# Autodesk Inventor assembly: 100027
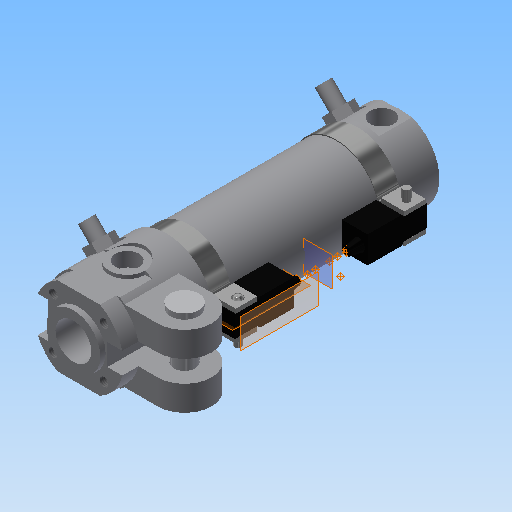
[picture p0: Inventor's stored thumbnail of the model, 512x512]
Saved by Autodesk Inventor 2020.1 (Build 241239000, 239)
## iProperties
Company: AUTODESK, INC.
Part Number: 100027
Document SubType Name: Assembly
Created: 2003-06-25
Designer: SCHNEIDER K.
Description: 70mm STROKE
Project: ADSK-000-000000
Control State: 0
Master: False
Checked Out: False
Shininess: 64.0
Length Units: 11269
Angle Units: 11279
Time Units: 11290
Mass Units: 11283
Length Display Precision: 2
Angle Display Precision: 2
Compacted: True
Stroke: 70.00 mm
Density: 0.0
Volumn: 0.0
Area: 0.0
PropertySet Name: Model Information
Title: PH CYLINDER
Author: schneik
Revision Number: -
## Documents named in this file (5)
- C:\Users\thom_tremblay\Desktop\Inventor ACP Data\Assemblies\PH-000-001.iam
- C:\Users\thom_tremblay\Desktop\Inventor ACP Data\Parts\PH-200-012.ipt
- C:\Users\thom_tremblay\Desktop\Inventor ACP Data\Parts\PH-200-010.ipt
- C:\Users\thom_tremblay\Desktop\Inventor ACP Data\Parts\PH-200-011.ipt
- C:\Users\thom_tremblay\Desktop\Inventor ACP Data\Parts\PH-200-014.ipt
## Components (6 placed, 4 different names)
1. PH-200-012:1 — Insert:6, Insert:7, Insert:4, Angle:4, Angle:5
2. PH-200-010:1 — Insert:1, Angle:1, Flush:1, Flush:2, Flush:3
3. PH-200-010:2 — Insert:2, Angle:2
4. PH-200-011:1 — Insert:6, Insert:1, Angle:1, Angle:4
5. PH-200-011:2 — Insert:7, Insert:2, Angle:2, Angle:5
6. PH-200-014:1 — Insert:4
## Relationships (15: Insert 5, Angle 4, Flush 3, Mate 3)
- Insert:6 (0.5 mm): PH-200-012:1 ↔ PH-200-011:1
- Insert:7 (23.5 mm): PH-200-012:1 ↔ PH-200-011:2
- Insert:1: PH-200-010:1 ↔ PH-200-011:1
- Angle:1 (0 deg): PH-200-010:1 ↔ PH-200-011:1
- Insert:2: PH-200-010:2 ↔ PH-200-011:2
- Angle:2 (0 deg): PH-200-010:2 ↔ PH-200-011:2
- Insert:4: PH-200-012:1 ↔ PH-200-014:1
- Angle:4 (180 deg): PH-200-012:1 ↔ PH-200-011:1
- Angle:5 (180 deg): PH-200-012:1 ↔ PH-200-011:2
- Flush:1 (20.5 mm): PH-200-010:1
- Flush:2 (5 mm): PH-200-010:1
- Flush:3 (-8 mm): PH-200-010:1
- Mate:2
- Mate:3
- Mate:4
